# Autodesk Inventor assembly: Mini V Carriage v2
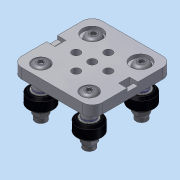
[picture p0: Inventor's stored thumbnail of the model, 180x180]
Saved by Autodesk Inventor 2013 (Build 170138000, 138)
## iProperties
Created: 2013-06-21
Part Number: Mini V Carriage v2
Document SubType Name: Assembly
Designer: Jon Hollander
Author: Jon Hollander
## Documents named in this file (8)
- D:\Dropbox\Research\Loom\Loom Vault\PoC V2\Library Parts\Mini V Carriage\Mini V Carriage v2.iam
- C:\Users\Work\Documents\Inventor\Content Center Files\R2013\en-US\Micro V Plate\Micro V Plate-Micro V Plate.ipt
- C:\Users\Work\Documents\Inventor\Content Center Files\R2013\en-US\Normal M5 Wheel Spacer\Normal M5 Wheel Spacer.ipt
- C:\Users\Work\Documents\Inventor\Content Center Files\R2013\en-US\Eccentric M5 Spacer\Eccentric M5 Spacer.ipt
- D:\Dropbox\Research\Loom\Loom Vault\Libary Import\Mini V Carriage\Mini Wheel and Bearings.iam
- C:\Users\Work\Documents\Inventor\Content Center Files\R2013\en-US\Micro V Precision Shim\Micro V Precision Shim.ipt
- C:\Users\Work\Documents\Inventor\Content Center Files\R2013\en-US\ANSI B18.3.4M(1)\ANSI B18.3.4M - M5 x 0.8 x 25(2).ipt
- C:\Users\Work\Documents\Inventor\Content Center Files\R2013\en-US\ANSI B18.16.3M(2)\ANSI B18.16.3M - Property Class 9 - Metric M5 x 0.8 Top Insert Type.ipt
## Components (21 placed, 7 different names)
1. Micro V Plate Micro V Plate:1 — Mate:11, Mate:13, Mate:14, Mate:17, Mate:18, Mate:21, Flush:1
2. Broached Hexagon Socket Button Head Cap Screw - Metric M5 x 0.8 x 25:1
3. Broached Hexagon Socket Button Head Cap Screw - Metric M5 x 0.8 x 25:2 — Mate:60
4. Broached Hexagon Socket Button Head Cap Screw - Metric M5 x 0.8 x 25:3
5. Broached Hexagon Socket Button Head Cap Screw - Metric M5 x 0.8 x 25:4
6. Normal M5 Wheel Spacer Normal M5 Wheel Spacer:1 — Mate:21, Mate:32
7. Normal M5 Wheel Spacer Normal M5 Wheel Spacer:2 — Mate:11, Mate:24
8. Eccentric M5 Spacer Eccentric M5 Spacer:1 — Mate:13, Mate:14, Mate:30
9. Eccentric M5 Spacer Eccentric M5 Spacer:2 — Mate:17, Mate:18, Mate:28
10. Mini Wheel and Bearings:1 [sub-assembly] — Mate:39, Flush:2, Mate:61
11. Mini Wheel and Bearings:2 [sub-assembly] — Mate:37, Mate:59
12. Mini Wheel and Bearings:3 [sub-assembly] — Mate:38, Mate:62
13. Mini Wheel and Bearings:4 [sub-assembly] — Mate:25, Mate:58
14. Micro V Precision Shim Micro V Precision Shim:1 — Mate:24, Mate:25
15. Micro V Precision Shim Micro V Precision Shim:3 — Mate:28, Mate:39
16. Micro V Precision Shim Micro V Precision Shim:4 — Mate:30, Mate:38
17. Micro V Precision Shim Micro V Precision Shim:5 — Mate:32, Mate:37
18. Prevailing Torque Type Hex Nut - Steel Metric Property Class 9 - Metric M5 x 0.8 Top Insert Type:1 — Mate:58
19. Prevailing Torque Type Hex Nut - Steel Metric Property Class 9 - Metric M5 x 0.8 Top Insert Type:2 — Mate:62
20. Prevailing Torque Type Hex Nut - Steel Metric Property Class 9 - Metric M5 x 0.8 Top Insert Type:3 — Mate:61
21. Prevailing Torque Type Hex Nut - Steel Metric Property Class 9 - Metric M5 x 0.8 Top Insert Type:4 — Mate:59, Mate:60
## Relationships (43: Mate 41, Flush 2)
- [Mate]: Micro V Plate Micro V Plate:1 ↔ Broached Hexagon Socket Button Head Cap Screw - Metric M5 x 0.8 x 25:1
- [Mate]: Micro V Plate Micro V Plate:1 ↔ Broached Hexagon Socket Button Head Cap Screw - Metric M5 x 0.8 x 25:2
- [Mate]: Micro V Plate Micro V Plate:1 ↔ Broached Hexagon Socket Button Head Cap Screw - Metric M5 x 0.8 x 25:3
- [Mate]: Micro V Plate Micro V Plate:1 ↔ Broached Hexagon Socket Button Head Cap Screw - Metric M5 x 0.8 x 25:4
- [Mate]: Broached Hexagon Socket Button Head Cap Screw - Metric M5 x 0.8 x 25:1 ↔ Normal M5 Wheel Spacer Normal M5 Wheel Spacer:2
- Mate:11: Micro V Plate Micro V Plate:1 ↔ Normal M5 Wheel Spacer Normal M5 Wheel Spacer:2
- Mate:13: Micro V Plate Micro V Plate:1 ↔ Eccentric M5 Spacer Eccentric M5 Spacer:1
- Mate:14: Micro V Plate Micro V Plate:1 ↔ Eccentric M5 Spacer Eccentric M5 Spacer:1
- [Mate]: Broached Hexagon Socket Button Head Cap Screw - Metric M5 x 0.8 x 25:3 ↔ Eccentric M5 Spacer Eccentric M5 Spacer:1
- [Mate]: Micro V Plate Micro V Plate:1 ↔ Broached Hexagon Socket Button Head Cap Screw - Metric M5 x 0.8 x 25:2
- Mate:17: Micro V Plate Micro V Plate:1 ↔ Eccentric M5 Spacer Eccentric M5 Spacer:2
- Mate:18: Micro V Plate Micro V Plate:1 ↔ Eccentric M5 Spacer Eccentric M5 Spacer:2
- [Mate]: Broached Hexagon Socket Button Head Cap Screw - Metric M5 x 0.8 x 25:4 ↔ Eccentric M5 Spacer Eccentric M5 Spacer:2
- [Mate]: Broached Hexagon Socket Button Head Cap Screw - Metric M5 x 0.8 x 25:2 ↔ Normal M5 Wheel Spacer Normal M5 Wheel Spacer:1
- Mate:21: Micro V Plate Micro V Plate:1 ↔ Normal M5 Wheel Spacer Normal M5 Wheel Spacer:1
- [Mate]: Broached Hexagon Socket Button Head Cap Screw - Metric M5 x 0.8 x 25:1 ↔ Mini Wheel and Bearings:4
- [Mate]: Broached Hexagon Socket Button Head Cap Screw - Metric M5 x 0.8 x 25:1 ↔ Micro V Precision Shim Micro V Precision Shim:1
- Mate:24: Normal M5 Wheel Spacer Normal M5 Wheel Spacer:2 ↔ Micro V Precision Shim Micro V Precision Shim:1
- Mate:25: Mini Wheel and Bearings:4 ↔ Micro V Precision Shim Micro V Precision Shim:1
- Mate:28: Eccentric M5 Spacer Eccentric M5 Spacer:2 ↔ Micro V Precision Shim Micro V Precision Shim:3
- [Mate]: Broached Hexagon Socket Button Head Cap Screw - Metric M5 x 0.8 x 25:4 ↔ Micro V Precision Shim Micro V Precision Shim:3
- Mate:30: Eccentric M5 Spacer Eccentric M5 Spacer:1 ↔ Micro V Precision Shim Micro V Precision Shim:4
- [Mate]: Broached Hexagon Socket Button Head Cap Screw - Metric M5 x 0.8 x 25:3 ↔ Micro V Precision Shim Micro V Precision Shim:4
- Mate:32: Normal M5 Wheel Spacer Normal M5 Wheel Spacer:1 ↔ Micro V Precision Shim Micro V Precision Shim:5
- [Mate]: Broached Hexagon Socket Button Head Cap Screw - Metric M5 x 0.8 x 25:2 ↔ Micro V Precision Shim Micro V Precision Shim:5
- [Mate]: Broached Hexagon Socket Button Head Cap Screw - Metric M5 x 0.8 x 25:2 ↔ Mini Wheel and Bearings:2
- [Mate]: Broached Hexagon Socket Button Head Cap Screw - Metric M5 x 0.8 x 25:3 ↔ Mini Wheel and Bearings:3
- [Mate]: Broached Hexagon Socket Button Head Cap Screw - Metric M5 x 0.8 x 25:4 ↔ Mini Wheel and Bearings:1
- Mate:37: Mini Wheel and Bearings:2 ↔ Micro V Precision Shim Micro V Precision Shim:5
- Mate:38: Mini Wheel and Bearings:3 ↔ Micro V Precision Shim Micro V Precision Shim:4
- Mate:39: Mini Wheel and Bearings:1 ↔ Micro V Precision Shim Micro V Precision Shim:3
- Flush:1 (-25 mm): Micro V Plate Micro V Plate:1
- Flush:2 (-4.4 mm): Mini Wheel and Bearings:1
- [Mate]: Broached Hexagon Socket Button Head Cap Screw - Metric M5 x 0.8 x 25:2 ↔ Prevailing Torque Type Hex Nut - Steel Metric Property Class 9 - Metric M5 x 0.8 Top Insert Type:4
- Mate:58: Mini Wheel and Bearings:4 ↔ Prevailing Torque Type Hex Nut - Steel Metric Property Class 9 - Metric M5 x 0.8 Top Insert Type:1
- Mate:59: Mini Wheel and Bearings:2 ↔ Prevailing Torque Type Hex Nut - Steel Metric Property Class 9 - Metric M5 x 0.8 Top Insert Type:4
- Mate:60: Broached Hexagon Socket Button Head Cap Screw - Metric M5 x 0.8 x 25:2 ↔ Prevailing Torque Type Hex Nut - Steel Metric Property Class 9 - Metric M5 x 0.8 Top Insert Type:4
- Mate:61: Mini Wheel and Bearings:1 ↔ Prevailing Torque Type Hex Nut - Steel Metric Property Class 9 - Metric M5 x 0.8 Top Insert Type:3
- Mate:62: Mini Wheel and Bearings:3 ↔ Prevailing Torque Type Hex Nut - Steel Metric Property Class 9 - Metric M5 x 0.8 Top Insert Type:2
- [Mate]: Micro V Plate Micro V Plate:1 ↔ Broached Hexagon Socket Button Head Cap Screw - Metric M5 x 0.8 x 25:1
- [Mate]: Broached Hexagon Socket Button Head Cap Screw - Metric M5 x 0.8 x 25:1 ↔ Prevailing Torque Type Hex Nut - Steel Metric Property Class 9 - Metric M5 x 0.8 Top Insert Type:1
- [Mate]: Broached Hexagon Socket Button Head Cap Screw - Metric M5 x 0.8 x 25:3 ↔ Prevailing Torque Type Hex Nut - Steel Metric Property Class 9 - Metric M5 x 0.8 Top Insert Type:2
- [Mate]: Broached Hexagon Socket Button Head Cap Screw - Metric M5 x 0.8 x 25:4 ↔ Prevailing Torque Type Hex Nut - Steel Metric Property Class 9 - Metric M5 x 0.8 Top Insert Type:3
